# Autodesk Inventor assembly: The Bump
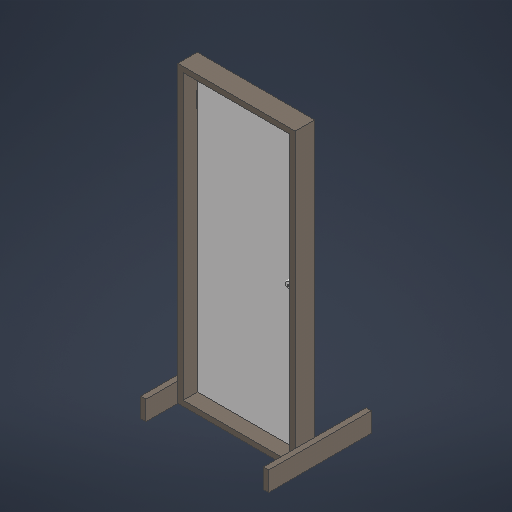
[picture p0: Inventor's stored thumbnail of the model, 512x512]
Saved by Autodesk Inventor 2026.2 (Build 302298000, 298)
## iProperties
Created: 2026-03-06
Part Number: The Bump
Document SubType Name: Assembly
Designer: brand
Author: brand
## Documents named in this file (6)
- C:\Users\brand\MMAE432\TheBump\The Bump.iam
- C:\Users\brand\MMAE432\TheBump\1518A15_Single Door\1518A15_Single Door\1518A15_Single Door.ipt
- C:\Users\brand\MMAE432\TheBump\DoorFrame.ipt
- C:\Users\brand\MMAE432\TheBump\1494A43_Mortise-Mount Entry Door Template Hinge\1494A43_Mortise-Mount Entry Door Template Hinge\1494A43_Mortise-Mount Entry Door Template Hinge.ipt
- C:\Users\brand\MMAE432\TheBump\DoorFrameBase.ipt
- C:\Users\brand\MMAE432\TheBump\12895A21_Door Knob\12895A21_Door Knob\12895A21_Door Knob.ipt
## Components (7 placed, 5 different names)
1. 1518A15_Single Door:1 — Mate:2, Mate:3, Mate:4, Flush:10, Mate:5, Flush:13
2. DoorFrame:1 — Flush:4, Flush:5, Mate:1, Flush:8, Mate:6, Flush:12
3. DoorFrameBase:1 — Flush:4, Flush:5, Flush:7, Flush:9
4. DoorFrameBase:2 — Flush:7, Mate:1, Flush:8, Flush:9
5. 12895A21_Door Knob:1 — Mate:2, Mate:3, Mate:4
6. 1494A43_Mortise-Mount Entry Door Template Hinge:6 — Flush:10, Mate:5, Flush:11, Flush:13, Cylindrical:1
7. 1494A43_Mortise-Mount Entry Door Template Hinge:7 — Mate:6, Flush:11, Flush:12, Cylindrical:1
## Relationships (16: Flush 9, Mate 6, CylindricalJoint 1)
- Flush:4: DoorFrame:1 ↔ DoorFrameBase:1
- Flush:5: DoorFrame:1 ↔ DoorFrameBase:1
- Flush:7: DoorFrameBase:1 ↔ DoorFrameBase:2
- Mate:1: DoorFrame:1 ↔ DoorFrameBase:2
- Flush:8: DoorFrame:1 ↔ DoorFrameBase:2
- Flush:9: DoorFrameBase:1 ↔ DoorFrameBase:2
- Mate:2: 1518A15_Single Door:1 ↔ 12895A21_Door Knob:1
- Mate:3: 1518A15_Single Door:1 ↔ 12895A21_Door Knob:1
- Mate:4 (15.7226 mm): 1518A15_Single Door:1 ↔ 12895A21_Door Knob:1
- Flush:10 (152.4 mm): 1518A15_Single Door:1 ↔ 1494A43_Mortise-Mount Entry Door Template Hinge:6
- Mate:5: 1518A15_Single Door:1 ↔ 1494A43_Mortise-Mount Entry Door Template Hinge:6
- Mate:6: DoorFrame:1 ↔ 1494A43_Mortise-Mount Entry Door Template Hinge:7
- Flush:11: 1494A43_Mortise-Mount Entry Door Template Hinge:6 ↔ 1494A43_Mortise-Mount Entry Door Template Hinge:7
- Flush:12: DoorFrame:1 ↔ 1494A43_Mortise-Mount Entry Door Template Hinge:7
- Flush:13: 1518A15_Single Door:1 ↔ 1494A43_Mortise-Mount Entry Door Template Hinge:6
- Cylindrical:1: 1494A43_Mortise-Mount Entry Door Template Hinge:6 ↔ 1494A43_Mortise-Mount Entry Door Template Hinge:7
